# Autodesk Inventor assembly: connecting_shaft
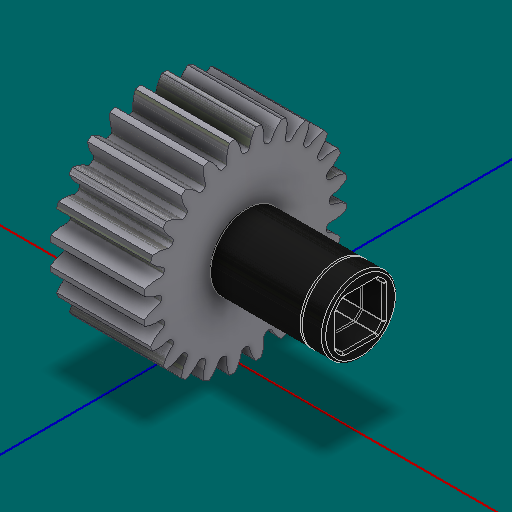
[picture p0: Inventor's stored thumbnail of the model, 512x512]
Saved by Autodesk Inventor 2025 (Build 290162000, 162)
## iProperties
Created: 2024-08-19
Part Number: connecting_shaft
Document SubType Name: Assembly
Designer: averey
Author: averey
## Documents named in this file (6)
- C:\Users\avere\vex_robotics_high_stakes\hardware\cad\ATLAS\tower\intake_gearbox\connecting_shaft.iam
- C:\Users\avere\vex_robotics_high_stakes\hardware\cad\VEX-CAD-Inventor\Motion\Gears\HS Gear\HS 24T Gear, No Insert.iam
- C:\Users\avere\vex_robotics_high_stakes\hardware\cad\VEX-CAD-Inventor\Motion\Gears\HS Gear.iam
- C:\Users\avere\vex_robotics_high_stakes\hardware\cad\VEX-CAD-Inventor\Motion\Shaft HS\HS Spacer\HSpacer .1250.ipt
- C:\Users\avere\vex_robotics_high_stakes\hardware\cad\VEX-CAD-Inventor\Motion\Shaft HS\HS Spacer.ipt
- C:\Users\avere\vex_robotics_high_stakes\hardware\cad\VEX-CAD-Inventor\Motion\Shaft HS\HS Spacer\HSpacer .5000.ipt
## Components (3 placed, 3 different names)
1. HS 24T Gear, No Insert:1 [sub-assembly] — Insert:2
2. HSpacer .1250:1 — Insert:1
3. HSpacer .5000:2 — Insert:1, Insert:2
## Relationships (2: Insert 2)
- Insert:1: HSpacer .1250:1 ↔ HSpacer .5000:2
- Insert:2: HS 24T Gear, No Insert:1 ↔ HSpacer .5000:2
